# Autodesk Inventor assembly: Individual Hook
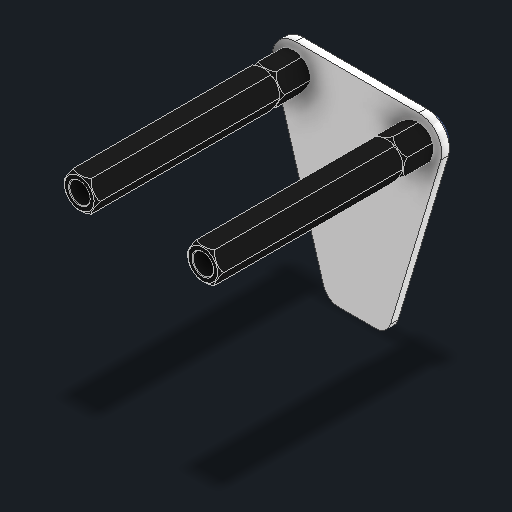
[picture p0: Inventor's stored thumbnail of the model, 512x512]
Saved by Autodesk Inventor 2025.1 (Build 291241000, 241)
## iProperties
Created: 2024-10-22
Part Number: Individual Hook
Document SubType Name: Assembly
Designer: averey
Author: averey
## Documents named in this file (7)
- C:\Users\avere\VEX\High Stakes\CAD\V3\Intake\Conveyer\Individual Hook.iam
- C:\Users\avere\VEX\High Stakes\CAD\V3\Intake\Conveyer\Custom Parts\Hook Gusset.ipt
- C:\Users\avere\VEX\High Stakes\CAD\ROBOPROS-CAD-Inventor\Structure\Standoff\Standoff .25.ipt
- C:\Users\avere\VEX\High Stakes\CAD\ROBOPROS-CAD-Inventor\Structure\Standoff.ipt
- C:\Users\avere\VEX\High Stakes\CAD\ROBOPROS-CAD-Inventor\Structure\Hardware\Screw Shoulder Robosource\SScrew Shoulder Smooth .500 x .04.ipt
- C:\Users\avere\VEX\High Stakes\CAD\ROBOPROS-CAD-Inventor\Structure\Hardware\Screw Shoulder Robosource.ipt
- C:\Users\avere\VEX\High Stakes\CAD\ROBOPROS-CAD-Inventor\Structure\Standoff\Standoff 1.50.ipt
## Components (7 placed, 4 different names)
1. Hook Gusset:1 — Mate:3
2. Standoff .25:1
3. Standoff .25:2
4. SScrew Shoulder Smooth .500 x .04:1
5. SScrew Shoulder Smooth .500 x .04:2
6. Standoff 1.50:4
7. Standoff 1.50:6
## Relationships (8: Insert 6, Mate 2)
- [Insert]: Hook Gusset:1 ↔ Standoff .25:1
- [Insert]: Hook Gusset:1 ↔ SScrew Shoulder Smooth .500 x .04:2
- [Insert]: Hook Gusset:1 ↔ SScrew Shoulder Smooth .500 x .04:1
- [Mate]: Standoff .25:2 ↔ SScrew Shoulder Smooth .500 x .04:2
- [Insert]: Hook Gusset:1 ↔ Standoff .25:2
- [Insert]: Standoff .25:2 ↔ Standoff 1.50:6
- [Insert]: Standoff .25:1 ↔ Standoff 1.50:4
- Mate:3 (-22.225 mm): Hook Gusset:1
## Named parameters: d19_d5 = 0 mm, d20_d6 = 0 mm, d21_d7 = 0 mm
